# Autodesk Inventor assembly: vehicle assembly v3
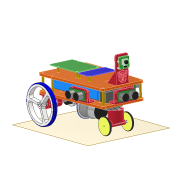
[picture p0: Inventor's stored thumbnail of the model, 180x180]
Saved by Autodesk Inventor 2022 (Build 260153000, 153)
## iProperties
Created: 2024-06-06
Part Number: vehicle assembly v3
Document SubType Name: Assembly
Designer: david
Author: david
## Documents named in this file (33)
- C:\Users\david\OneDrive\Documents\Inventor\WRO_FE_2024\vehicle assembly v3.iam
- C:\Users\david\OneDrive\Documents\Inventor\WRO_FE_2024\base plate.ipt
- C:\Users\david\OneDrive\Documents\Inventor\WRO_FE_2024\bearing holder.ipt
- C:\Users\david\OneDrive\Documents\Inventor\WRO_FE_2024\rear shaft.ipt
- rear shaft.ipt
- C:\Users\david\OneDrive\Documents\Inventor\WRO_FE_2024\rear wheel.ipt
- rear wheel.ipt
- C:\Users\david\OneDrive\Documents\Inventor\WRO_FE_2024\servo motor HS-7955TG.iam
- C:\Users\david\OneDrive\Documents\Inventor\WRO_FE_2024\steering.ipt
- C:\Users\david\OneDrive\Documents\Inventor\WRO_FE_2024\dfifferential.ipt
- C:\Users\david\OneDrive\Documents\Inventor\WRO_FE_2024\front shaft.ipt
- C:\Users\david\OneDrive\Documents\Inventor\WRO_FE_2024\front wheel.ipt
- C:\Users\david\OneDrive\Documents\Inventor\WRO_FE_2024\hobby motor mount.ipt
- C:\Users\david\OneDrive\Documents\Inventor\WRO_FE_2024\DC Hobby Motor.ipt
- C:\Users\david\OneDrive\Documents\Inventor\WRO_FE_2024\driver gear adapter.ipt
- C:\Users\david\OneDrive\Documents\Inventor\WRO_FE_2024\driver gear.ipt
- C:\Users\david\OneDrive\Documents\Inventor\WRO_FE_2024\rear wheel 86mm.ipt
- C:\Users\david\OneDrive\Documents\Inventor\WRO_FE_2024\rear shaft v2.ipt
- C:\Users\david\OneDrive\Documents\Inventor\WRO_FE_2024\12v DC motor mount.ipt
- C:\Users\david\OneDrive\Documents\Inventor\WRO_FE_2024\12v DC motor.ipt
- C:\Users\david\OneDrive\Documents\Inventor\WRO_FE_2024\front shaft v2.ipt
- C:\Users\david\OneDrive\Documents\Inventor\WRO_FE_2024\driver gear adapter v2.ipt
- C:\Users\david\OneDrive\Documents\Inventor\WRO_FE_2024\stand M3-L10.ipt
- C:\Users\david\OneDrive\Documents\Inventor\WRO_FE_2024\top plate.ipt
- C:\Users\david\OneDrive\Documents\Inventor\WRO_FE_2024\raspberry pi.ipt
- C:\Users\david\OneDrive\Documents\Inventor\WRO_FE_2024\3s lipo battery.ipt
- C:\Users\david\OneDrive\Documents\Inventor\WRO_FE_2024\ultrasonic mount.ipt
- C:\Users\david\OneDrive\Documents\Inventor\WRO_FE_2024\US-015.ipt
- C:\Users\david\OneDrive\Documents\Inventor\WRO_FE_2024\stand M3-L30.ipt
- C:\Users\david\OneDrive\Documents\Inventor\WRO_FE_2024\LM2596 Buck Converter.ipt
- C:\Users\david\OneDrive\Documents\Inventor\WRO_FE_2024\camera mount.ipt
- C:\Users\david\OneDrive\Documents\Inventor\WRO_FE_2024\raspberry pi camera v2.ipt
- C:\Users\david\OneDrive\Documents\Inventor\WRO_FE_2024\stub.ipt
## Components (57 placed, 34 different names)
1. raspberry pi:2 — Insert:58, Insert:59
2. base plate:1 — Insert:60, Insert:61, Insert:62, Insert:63, Mate:9, Mate:10, Insert:72, Insert:73, Mate:11, Flush:6, Flush:7, Flush:8, Insert:74, Insert:75, Mate:12, Flush:9, Insert:128, Insert:129, Insert:130, Insert:131, Insert:132, Insert:133, Insert:134, Insert:135, Insert:136, Insert:137, Insert:138, Insert:139, Insert:140, Insert:141
3. top plate:1 — Insert:52, Insert:53, Insert:54, Insert:55, Insert:56, Insert:57, Insert:76, Insert:108, Insert:109, Insert:110, Insert:111, Insert:126, Insert:127
4. bearing holder:1 — Insert:138, Insert:139, Insert:142
5. bearing holder:2 — Insert:140, Insert:141
6. bearing holder:3 — Insert:136, Insert:137
7. bearing holder:4 — Insert:134, Insert:135, Insert:143
8. dfifferential:1 — Insert:77, Insert:78
9. driver gear:1 — Insert:29, Insert:47
10. rear shaft:right — Angle:1, Insert:78, Insert:79, Angle:6
11. rear shaft:left — Angle:2, Insert:77, Angle:7, Insert:80
12. rear shaft v2: right — Insert:83, Angle:9, Insert:143
13. rear shaft v2: left — Insert:84, Angle:8, Insert:142
14. rear wheel:right — Insert:79, Angle:6
15. rear wheel:left — Angle:7, Insert:80
16. rear wheel 86mm: right — Insert:83, Angle:9
17. rear wheel 86mm: left — Tangent:1, Insert:84, Angle:8
18. hobby motor mount:1 — Insert:25, Insert:26
19. DC Hobby Motor:1 — Insert:25, Insert:26, Insert:28
20. driver gear adapter:1 — Insert:28, Insert:29
21. 12v DC motor mount:1 — Insert:38, Insert:39, Insert:72, Insert:73
22. 12v DC motor:1 — Insert:38, Insert:39, Insert:46, Angle:5
23. driver gear adapter v2:1 — Insert:46, Insert:47, Angle:5
24. servo motor HS-7955TG:1 [sub-assembly] — Mate:2, Insert:20, Mate:9, Mate:10, Mate:11
25. steering:1 — Insert:20, Steering Angle, Mate:8, Flush:5
26. front wheel:1 — Insert:35, Insert:43, Angle:11
27. front wheel:2 — Insert:34, Insert:42, Angle:10
28. front shaft:1 — Flush:4, Insert:34, Insert:35
29. front shaft v2:1 — Mate:8, Insert:42, Insert:43, Flush:5, Angle:10, Angle:11
30. stand M3-L30:2 — Insert:60
31. stand M3-L30:3 — Insert:53, Insert:63
32. stand M3-L30:1 — Insert:52, Insert:61
33. stand M3-L30:4 — Insert:62
34. stand M3-L30:9 — Insert:74
35. stand M3-L30:10 — Insert:75, Insert:76
36. stand M3-L10:1 — Insert:55
37. stand M3-L10:2 — Insert:57
38. stand M3-L10:3 — Insert:54, Insert:59
39. stand M3-L10:4 — Insert:56, Insert:58
40. 3s lipo battery:1 — Mate:12, Flush:9, Flush:10
41. ultrasonic mount:1 — Insert:102, Insert:103, Insert:128, Insert:129
42. US-015:1 — Insert:102, Insert:103
43. ultrasonic mount:2 — Insert:104, Insert:105, Insert:130, Insert:131
44. ultrasonic mount:3 — Insert:106, Insert:107, Insert:132, Insert:133
45. US-015:2 — Insert:106, Insert:107
46. US-015:3 — Insert:104, Insert:105
47. LM2596 Buck Converter:1 — Insert:112, Insert:113
48. stand M3-L10:5 — Insert:109
49. stand M3-L10:6 — Insert:111
50. stand M3-L10:7 — Insert:108, Insert:112
51. stand M3-L10:8 — Insert:110, Insert:113
52. camera mount:1 — Insert:124, Insert:125, Insert:126, Insert:127
53. raspberry pi camera v2:1 — Insert:120, Insert:121, Insert:122, Insert:123
54. stub:1 — Insert:123
55. stub:2 — Insert:121, Insert:124
56. stub:3 — Insert:122
57. stub:4 — Insert:120, Insert:125
## Relationships (97: Insert 72, Angle 11, Flush 7, Mate 6, Tangent 1)
- Angle:1 (0 deg): rear shaft:right
- Angle:2 (0 deg): rear shaft:left
- Mate:2: servo motor HS-7955TG:1
- Insert:20: servo motor HS-7955TG:1 ↔ steering:1
- Steering Angle [Angle] (0 deg): steering:1
- Insert:25: hobby motor mount:1 ↔ DC Hobby Motor:1
- Insert:26: hobby motor mount:1 ↔ DC Hobby Motor:1
- Insert:28: DC Hobby Motor:1 ↔ driver gear adapter:1
- Insert:29: driver gear:1 ↔ driver gear adapter:1
- Flush:4: front shaft:1
- Insert:34: front wheel:2 ↔ front shaft:1
- Insert:35: front wheel:1 ↔ front shaft:1
- Angle:4 (0 deg)
- Tangent:1: rear wheel 86mm: left
- Insert:38: 12v DC motor mount:1 ↔ 12v DC motor:1
- Insert:39: 12v DC motor mount:1 ↔ 12v DC motor:1
- Mate:8: steering:1 ↔ front shaft v2:1
- Insert:42: front wheel:2 ↔ front shaft v2:1
- Insert:43: front wheel:1 ↔ front shaft v2:1
- Insert:46: 12v DC motor:1 ↔ driver gear adapter v2:1
- Insert:47: driver gear:1 ↔ driver gear adapter v2:1
- Flush:5: steering:1 ↔ front shaft v2:1
- Angle:5 (180 deg): 12v DC motor:1 ↔ driver gear adapter v2:1
- Insert:52: top plate:1 ↔ stand M3-L30:1
- Insert:53: top plate:1 ↔ stand M3-L30:3
- Insert:54: top plate:1 ↔ stand M3-L10:3
- Insert:55: top plate:1 ↔ stand M3-L10:1
- Insert:56: top plate:1 ↔ stand M3-L10:4
- Insert:57: top plate:1 ↔ stand M3-L10:2
- Insert:58: raspberry pi:2 ↔ stand M3-L10:4
- Insert:59: raspberry pi:2 ↔ stand M3-L10:3
- Insert:60: base plate:1 ↔ stand M3-L30:2
- Insert:61: base plate:1 ↔ stand M3-L30:1
- Insert:62: base plate:1 ↔ stand M3-L30:4
- Insert:63: base plate:1 ↔ stand M3-L30:3
- Mate:9: base plate:1 ↔ servo motor HS-7955TG:1
- Mate:10: base plate:1 ↔ servo motor HS-7955TG:1
- Insert:72: base plate:1 ↔ 12v DC motor mount:1
- Insert:73: base plate:1 ↔ 12v DC motor mount:1
- Mate:11: base plate:1 ↔ servo motor HS-7955TG:1
- Flush:6: base plate:1
- Flush:7: base plate:1
- Flush:8: base plate:1
- Insert:74: base plate:1 ↔ stand M3-L30:9
- Insert:75: base plate:1 ↔ stand M3-L30:10
- Insert:76: top plate:1 ↔ stand M3-L30:10
- Insert:77: dfifferential:1 ↔ rear shaft:left
- Insert:78: dfifferential:1 ↔ rear shaft:right
- Insert:79: rear shaft:right ↔ rear wheel:right
- Angle:6 (0 deg): rear shaft:right ↔ rear wheel:right
- Angle:7 (0 deg): rear shaft:left ↔ rear wheel:left
- Insert:80: rear shaft:left ↔ rear wheel:left
- Insert:83: rear shaft v2: right ↔ rear wheel 86mm: right
- Insert:84: rear shaft v2: left ↔ rear wheel 86mm: left
- Angle:8 (180 deg): rear shaft v2: left ↔ rear wheel 86mm: left
- Angle:9 (180 deg): rear shaft v2: right ↔ rear wheel 86mm: right
- Mate:12: base plate:1 ↔ 3s lipo battery:1
- Flush:9: base plate:1 ↔ 3s lipo battery:1
- Flush:10: 3s lipo battery:1
- Angle:10 (0 deg): front wheel:2 ↔ front shaft v2:1
- Angle:11 (0 deg): front wheel:1 ↔ front shaft v2:1
- Insert:102: ultrasonic mount:1 ↔ US-015:1
- Insert:103: ultrasonic mount:1 ↔ US-015:1
- Insert:104: ultrasonic mount:2 ↔ US-015:3
- Insert:105: ultrasonic mount:2 ↔ US-015:3
- Insert:106: ultrasonic mount:3 ↔ US-015:2
- Insert:107: ultrasonic mount:3 ↔ US-015:2
- Insert:108: top plate:1 ↔ stand M3-L10:7
- Insert:109: top plate:1 ↔ stand M3-L10:5
- Insert:110: top plate:1 ↔ stand M3-L10:8
- Insert:111: top plate:1 ↔ stand M3-L10:6
- Insert:112: LM2596 Buck Converter:1 ↔ stand M3-L10:7
- Insert:113: LM2596 Buck Converter:1 ↔ stand M3-L10:8
- Insert:120: raspberry pi camera v2:1 ↔ stub:4
- Insert:121: raspberry pi camera v2:1 ↔ stub:2
- Insert:122: raspberry pi camera v2:1 ↔ stub:3
- Insert:123: raspberry pi camera v2:1 ↔ stub:1
- Insert:124: camera mount:1 ↔ stub:2
- Insert:125: camera mount:1 ↔ stub:4
- Insert:126: top plate:1 ↔ camera mount:1
- Insert:127: top plate:1 ↔ camera mount:1
- Insert:128: base plate:1 ↔ ultrasonic mount:1
- Insert:129: base plate:1 ↔ ultrasonic mount:1
- Insert:130: base plate:1 ↔ ultrasonic mount:2
- Insert:131: base plate:1 ↔ ultrasonic mount:2
- Insert:132: base plate:1 ↔ ultrasonic mount:3
- Insert:133: base plate:1 ↔ ultrasonic mount:3
- Insert:134: base plate:1 ↔ bearing holder:4
- Insert:135: base plate:1 ↔ bearing holder:4
- Insert:136: base plate:1 ↔ bearing holder:3
- Insert:137: base plate:1 ↔ bearing holder:3
- Insert:138: base plate:1 ↔ bearing holder:1
- Insert:139: base plate:1 ↔ bearing holder:1
- Insert:140: base plate:1 ↔ bearing holder:2
- Insert:141: base plate:1 ↔ bearing holder:2
- Insert:142: bearing holder:1 ↔ rear shaft v2: left
- Insert:143: bearing holder:4 ↔ rear shaft v2: right
